# Autodesk Inventor assembly: gear-smol
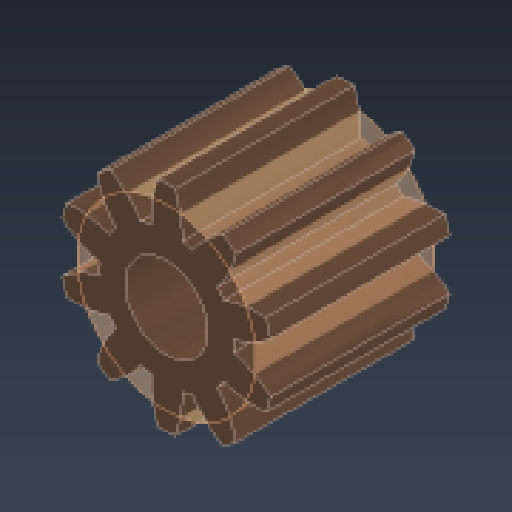
[picture p0: Inventor's stored thumbnail of the model, 512x512]
Saved by Autodesk Inventor 2023 (Build 270158000, 158)
## iProperties
Created: 2025-04-27
Part Number: gear-smol
Document SubType Name: Assembly
Designer: szymo
Surface Area: 2.24861 cm^2
Volume: 0.0775085 cm^3
Author: szymo
## Documents named in this file (2)
- D:\tech\robotyka\robots\evangelion-turbo\inventor-project\gear-smol.iam
- D:\tech\robotyka\robots\evangelion-turbo\inventor-project\gear-smol\Design Accelerator\Spur Gears1.iam
## Components (1 placed, 1 different names)
1. Spur Gears:1 [sub-assembly] — Mate:1, Mate:2, Flush:1, Angle:1, Angle:2, Angle:3
## Relationships (6: Angle 3, Mate 2, Flush 1)
- Mate:1: Spur Gears:1
- Mate:2: Spur Gears:1
- Flush:1: Spur Gears:1
- Angle:1 (180 deg): Spur Gears:1
- Angle:2 (180 deg): Spur Gears:1
- Angle:3 (0 deg): Spur Gears:1
